# Autodesk Inventor assembly: Trebuchet
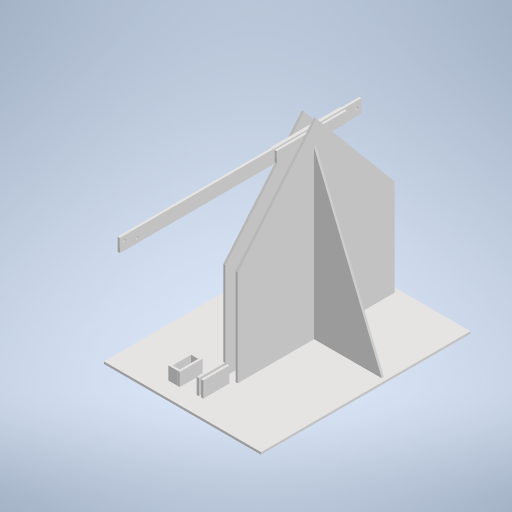
[picture p0: Inventor's stored thumbnail of the model, 512x512]
Saved by Autodesk Inventor 2023 (Build 270158000, 158)
## iProperties
Created: 2023-10-15
Part Number: Trebuchet
Document SubType Name: Assembly
Designer: Nate
Author: Nate
## Documents named in this file (10)
- C:\Users\Nate\Desktop\Trebuchet\Trebuchet.iam
- C:\Users\Nate\Desktop\Trebuchet\base.ipt
- C:\Users\Nate\Desktop\Trebuchet\side.ipt
- C:\Users\Nate\Desktop\Trebuchet\side support.ipt
- C:\Users\Nate\Desktop\Trebuchet\servo long side.ipt
- C:\Users\Nate\Desktop\Trebuchet\servo short side.ipt
- C:\Users\Nate\Desktop\Trebuchet\pin holder.ipt
- C:\Users\Nate\Desktop\Trebuchet\pin holder middle.ipt
- C:\Users\Nate\Desktop\Trebuchet\arm assembly.iam
- C:\Users\Nate\Desktop\Trebuchet\acrylic rod.ipt
## Components (14 placed, 9 different names)
1. base:1 — Mate:3, Mate:4, Flush:1, Mate:5, Mate:6, Mate:7, Mate:8, Mate:9, Mate:10, Mate:11, Rigid:3, Mate:12, Mate:13, Mate:14, Mate:15, Mate:16, Mate:17, Mate:18, Mate:19
2. side:1 — Mate:14, Mate:15, Mate:20
3. side:2 — Mate:12, Mate:13, Mate:21
4. side support:1 — Mate:18, Mate:19
5. side support:2 — Mate:16, Mate:17
6. servo long side:1 — Mate:3
7. servo long side:2 — Mate:4
8. servo short side:1 — Flush:1
9. servo short side:2 — Mate:5, Mate:6, Mate:7
10. pin holder:1 — Mate:8, Mate:9
11. pin holder:2 — Mate:10, Mate:11
12. pin holder middle:1 — Rigid:3
13. arm assembly:1 [sub-assembly] — Mate:20
14. acrylic rod:1 — Mate:21
## Relationships (21: Mate 19, Flush 1, WeldJoint 1)
- Mate:3: base:1 ↔ servo long side:1
- Mate:4: base:1 ↔ servo long side:2
- Flush:1: base:1 ↔ servo short side:1
- Mate:5: base:1 ↔ servo short side:2
- Mate:6: base:1 ↔ servo short side:2
- Mate:7: base:1 ↔ servo short side:2
- Mate:8: base:1 ↔ pin holder:1
- Mate:9: base:1 ↔ pin holder:1
- Mate:10: base:1 ↔ pin holder:2
- Mate:11: base:1 ↔ pin holder:2
- Rigid:3 [WeldJoint]: base:1 ↔ pin holder middle:1
- Mate:12: base:1 ↔ side:2
- Mate:13: base:1 ↔ side:2
- Mate:14: base:1 ↔ side:1
- Mate:15: base:1 ↔ side:1
- Mate:16: base:1 ↔ side support:2
- Mate:17: base:1 ↔ side support:2
- Mate:18: base:1 ↔ side support:1
- Mate:19: base:1 ↔ side support:1
- Mate:20 (6.35 mm): side:1 ↔ arm assembly:1
- Mate:21: side:2 ↔ acrylic rod:1
